# Autodesk Inventor assembly: ELB-ASM-1000
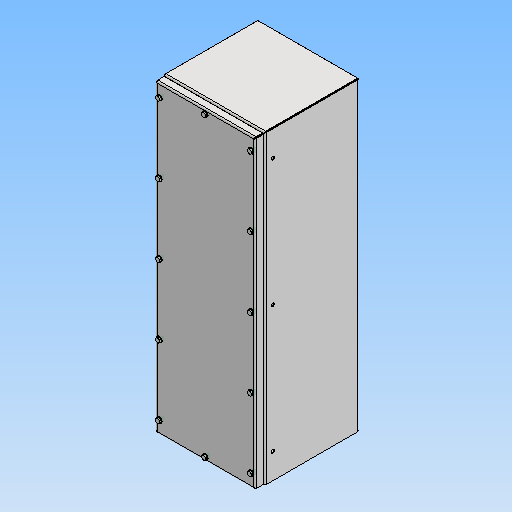
[picture p0: Inventor's stored thumbnail of the model, 512x512]
Saved by Autodesk Inventor 2025.4 (Build 294407000, 407)
## iProperties
Created: 2025-12-12
Part Number: ELB-ASM-1000
Document SubType Name: Assembly
Designer: josh
Description: ELECTRICAL ENCLOSURE 8" X 8" X 24"
Mass: 5756.02 g
Surface Area: 9698.82 cm^2
Volume: 733.251 cm^3
Density: 7.85 g/cm^3
Author: josh
## iProperties of the stored document MemberDocs/xIoy5laheBsymk5l0Pqjfjocp2c
Created: 2025-12-12
Part Number: ELB-ASM-1000
Document SubType Name: Assembly
Designer: josh
Mass: 7498.85 g
Surface Area: 12644.4 cm^2
Volume: 955.268 cm^3
Density: 7.85 g/cm^3
Author: josh
## iProperties of the stored document MemberDocs/xNeekpwlrHs1s0hkiGjj3irq5Wh
Created: 2025-12-12
Part Number: ELB-ASM-1000
Document SubType Name: Assembly
Designer: josh
Description: ELECTRICAL ENCLOSURE 8" X 8" X 24"
Author: josh
## Documents named in this file (11)
- R:\A1- Neuweg Design Data\OM Robotics\CLEANING ROBOT TOWER PROJECT\ELB-ASM-1000.iam
- R:\A1- Neuweg Design Data\OM Robotics\CLEANING ROBOT TOWER PROJECT\ELB-1002.ipt
- R:\A1- Neuweg Design Data\OM Robotics\CLEANING ROBOT TOWER PROJECT\ELB-1003.ipt
- R:\A1- Neuweg Design Data\OM Robotics\CLEANING ROBOT TOWER PROJECT\ELB-1004.ipt
- R:\A1- Neuweg Design Data\OM Robotics\CLEANING ROBOT TOWER PROJECT\ELB-1005.ipt
- R:\A1- Neuweg Design Data\OM Robotics\CLEANING ROBOT TOWER PROJECT\90096A324.ipt
- C:\WORK\INVENTOR PROJECTS\misc custom projects\O&M ROBOTICS\TOWER & ARM\ELB-1002.ipt
- C:\WORK\INVENTOR PROJECTS\misc custom projects\O&M ROBOTICS\TOWER & ARM\ELB-1003.ipt
- C:\WORK\INVENTOR PROJECTS\misc custom projects\O&M ROBOTICS\TOWER & ARM\ELB-1004.ipt
- C:\WORK\INVENTOR PROJECTS\misc custom projects\O&M ROBOTICS\TOWER & ARM\ELB-1005.ipt
- C:\WORK\INVENTOR PROJECTS\misc custom projects\O&M ROBOTICS\TOWER & ARM\90096A324\90096A324\90096A324.ipt
## Components (16 placed, 5 different names)
1. ELB-1002:1
2. ELB-1003:1
3. ELB-1004:1
4. ELB-1005:1 — Insert:1, Insert:2, Insert:3, Insert:4, Insert:5, Insert:6, Insert:7, Insert:8, Insert:9, Insert:10, Insert:11, Insert:12
5. 90096A324:1 — Insert:1
6. 90096A324:2 — Insert:2
7. 90096A324:3 — Insert:3
8. 90096A324:4 — Insert:4
9. 90096A324:5 — Insert:5
10. 90096A324:6 — Insert:6
11. 90096A324:7 — Insert:7
12. 90096A324:8 — Insert:8
13. 90096A324:9 — Insert:9
14. 90096A324:10 — Insert:10
15. 90096A324:11 — Insert:11
16. 90096A324:12 — Insert:12
## Relationships (12: Insert 12)
- Insert:1: ELB-1005:1 ↔ 90096A324:1
- Insert:2: ELB-1005:1 ↔ 90096A324:2
- Insert:3: ELB-1005:1 ↔ 90096A324:3
- Insert:4: ELB-1005:1 ↔ 90096A324:4
- Insert:5: ELB-1005:1 ↔ 90096A324:5
- Insert:6: ELB-1005:1 ↔ 90096A324:6
- Insert:7: ELB-1005:1 ↔ 90096A324:7
- Insert:8: ELB-1005:1 ↔ 90096A324:8
- Insert:9: ELB-1005:1 ↔ 90096A324:9
- Insert:10: ELB-1005:1 ↔ 90096A324:10
- Insert:11: ELB-1005:1 ↔ 90096A324:11
- Insert:12: ELB-1005:1 ↔ 90096A324:12
